# Autodesk Inventor assembly: Leadscrew Constraint Front for 4040 - Assembly
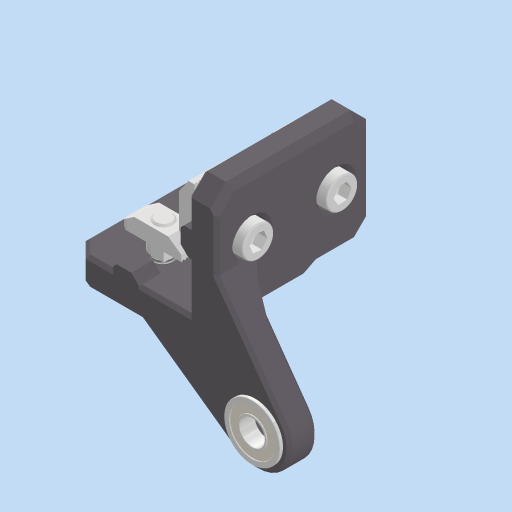
[picture p0: Inventor's stored thumbnail of the model, 512x512]
Saved by Autodesk Inventor 2023.2 (Build 272271000, 271)
## iProperties
Created: 2023-11-23
Part Number: Leadscrew Constraint Front for 4040 - Assembly
Document SubType Name: Assembly
Designer: Nils Bade
Author: Nils Bade
## Documents named in this file (6)
- C:\Users\nilsb\Documents\Inventor\Projektarbeit-Bade\RatRig_modified\Leadscrew Constraint Front for 4040 - Assembly.iam
- C:\Users\nilsb\Documents\Inventor\Projektarbeit-Bade\RatRig_modified\Leadscrew Constraint Front for 4040.ipt
- Leadscrew Constraint Front for 4040.ipt
- C:\Users\nilsb\Documents\Inventor\Projektarbeit-Bade\Schrauben\Cap Head Screw M6x16 - DIN912.ipt
- C:\Users\nilsb\Documents\Inventor\Projektarbeit-Bade\RatRig_modified\T-NUT - DropIn 4040 SERIES - M6.ipt
- C:\Users\nilsb\Documents\Inventor\Projektarbeit-Bade\RatRig_Standards\Ball Bearing - F688ZZ v1.ipt
## Components (10 placed, 4 different names)
1. Leadscrew Constraint Front for 4040:1 — Passend:1, Passend:2, Passend:3, Passend:4, Passend:5, Passend:6, Passend:7, Passend:8, Passend:13, Passend:14, Passend:15, Passend:16, Winkel:1, Winkel:2, Winkel:3, Winkel:4, Passend:17, Passend:18
2. Cap Head Screw M6x16 - DIN912:1 — Passend:3, Passend:5, Passend:9
3. Cap Head Screw M6x16 - DIN912:2 — Passend:4, Passend:6, Passend:10
4. Cap Head Screw M6x16 - DIN912:3 — Passend:1, Passend:7, Passend:11
5. Cap Head Screw M6x16 - DIN912:4 — Passend:2, Passend:8, Passend:12
6. T-NUT - DROP IN TYPE FOR 40 SERIES - M6:1 — Passend:9, Passend:15, Winkel:2
7. T-NUT - DROP IN TYPE FOR 40 SERIES - M6:2 — Passend:10, Passend:14, Winkel:4
8. T-NUT - DROP IN TYPE FOR 40 SERIES - M6:3 — Passend:11, Passend:16, Winkel:1
9. T-NUT - DROP IN TYPE FOR 40 SERIES - M6:4 — Passend:12, Passend:13, Winkel:3
10. Ball Bearing - F688ZZ v1:1 — Passend:17, Passend:18
## Relationships (22: Mate 18, Angle 4)
- Passend:1 [Mate]: Leadscrew Constraint Front for 4040:1 ↔ Cap Head Screw M6x16 - DIN912:3
- Passend:2 [Mate]: Leadscrew Constraint Front for 4040:1 ↔ Cap Head Screw M6x16 - DIN912:4
- Passend:3 [Mate]: Leadscrew Constraint Front for 4040:1 ↔ Cap Head Screw M6x16 - DIN912:1
- Passend:4 [Mate]: Leadscrew Constraint Front for 4040:1 ↔ Cap Head Screw M6x16 - DIN912:2
- Passend:5 [Mate]: Leadscrew Constraint Front for 4040:1 ↔ Cap Head Screw M6x16 - DIN912:1
- Passend:6 [Mate]: Leadscrew Constraint Front for 4040:1 ↔ Cap Head Screw M6x16 - DIN912:2
- Passend:7 [Mate]: Leadscrew Constraint Front for 4040:1 ↔ Cap Head Screw M6x16 - DIN912:3
- Passend:8 [Mate]: Leadscrew Constraint Front for 4040:1 ↔ Cap Head Screw M6x16 - DIN912:4
- Passend:9 [Mate]: Cap Head Screw M6x16 - DIN912:1 ↔ T-NUT - DROP IN TYPE FOR 40 SERIES - M6:1
- Passend:10 [Mate]: Cap Head Screw M6x16 - DIN912:2 ↔ T-NUT - DROP IN TYPE FOR 40 SERIES - M6:2
- Passend:11 [Mate]: Cap Head Screw M6x16 - DIN912:3 ↔ T-NUT - DROP IN TYPE FOR 40 SERIES - M6:3
- Passend:12 [Mate]: Cap Head Screw M6x16 - DIN912:4 ↔ T-NUT - DROP IN TYPE FOR 40 SERIES - M6:4
- Passend:13 [Mate] (5.5 mm): Leadscrew Constraint Front for 4040:1 ↔ T-NUT - DROP IN TYPE FOR 40 SERIES - M6:4
- Passend:14 [Mate] (5.5 mm): Leadscrew Constraint Front for 4040:1 ↔ T-NUT - DROP IN TYPE FOR 40 SERIES - M6:2
- Passend:15 [Mate] (5.5 mm): Leadscrew Constraint Front for 4040:1 ↔ T-NUT - DROP IN TYPE FOR 40 SERIES - M6:1
- Passend:16 [Mate] (5.5 mm): Leadscrew Constraint Front for 4040:1 ↔ T-NUT - DROP IN TYPE FOR 40 SERIES - M6:3
- Winkel:1 [Angle] (0 deg): Leadscrew Constraint Front for 4040:1 ↔ T-NUT - DROP IN TYPE FOR 40 SERIES - M6:3
- Winkel:2 [Angle] (0 deg): Leadscrew Constraint Front for 4040:1 ↔ T-NUT - DROP IN TYPE FOR 40 SERIES - M6:1
- Winkel:3 [Angle] (0 deg): Leadscrew Constraint Front for 4040:1 ↔ T-NUT - DROP IN TYPE FOR 40 SERIES - M6:4
- Winkel:4 [Angle] (0 deg): Leadscrew Constraint Front for 4040:1 ↔ T-NUT - DROP IN TYPE FOR 40 SERIES - M6:2
- Passend:17 [Mate]: Leadscrew Constraint Front for 4040:1 ↔ Ball Bearing - F688ZZ v1:1
- Passend:18 [Mate]: Leadscrew Constraint Front for 4040:1 ↔ Ball Bearing - F688ZZ v1:1
